# Autodesk Inventor assembly: Portalfraese_V2_Z-Axis
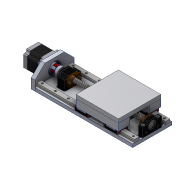
[picture p0: Inventor's stored thumbnail of the model, 180x180]
Saved by Autodesk Inventor 2016 (Build 200138000, 138)
## iProperties
Created: 2015-07-20
Part Number: Portalfraese_V2_Z-Axis
Document SubType Name: Assembly
Mass: 4544.64 g
Surface Area: 3288.98 cm^2
Volume: 1436.27 cm^3
Density: 3.16419 g/cm^3
## Documents named in this file (9)
- C:\Dropbox\Inventor\Projects\Portalfraese_V2_Z-Axis\Portalfraese_V2_Z-Axis.iam
- C:\Dropbox\Inventor\Projects\Portalfraese_V2_Z-Axis\Linearfuehrung Bosch Rexroth R0442.iam
- C:\Dropbox\Inventor\Projects\Portalfraese_V2_Z-Axis\ISSOKU_Ballscrew_D12x160_05_590104-13.iam
- C:\Dropbox\Inventor\Projects\Portalfraese_V2_Z-Axis\Grundplatte.ipt
- C:\Dropbox\Inventor\Projects\Portalfraese_V2_Z-Axis\Befestigungsplatte.ipt
- C:\Dropbox\Inventor\Projects\001_EK-Teile\Motor Nema 23.ipt
- C:\Dropbox\Inventor\Projects\Portalfraese_V2_Z-Axis\Motorhalterung.ipt
- C:\Dropbox\Inventor\Projects\Portalfraese_V2_Z-Axis\Distanzblock.ipt
- C:\Dropbox\Inventor\Projects\Portalfraese_V2_Z-Axis\Klauenkupplung.ipt
## Components (10 placed, 8 different names)
1. ISSOKU_Ballscrew_D12x160_05_590104-13:1 [sub-assembly] — Flush:1, Flush:2, Flush:6, Flush:7, Mate:3, Mate:5, Mate:6, Mate:7, Mate:8, Insert:1
2. Linearfuehrung Bosch Rexroth R0442:1 [sub-assembly] — Flush:1, Flush:3, Mate:1, Mate:2, Flush:4, Flush:5, Flush:6, Flush:7, Mate:4, Flush:8, Flush:9, Mate:12
3. Linearfuehrung Bosch Rexroth R0442:2 [sub-assembly] — Flush:2, Flush:3, Mate:2, Flush:4, Flush:5, Mate:13
4. Grundplatte:1 — Mate:3, Mate:4, Flush:8, Mate:5, Angle:1, Mate:10, Flush:10
5. Befestigungsplatte:1 — Mate:6, Flush:9, Mate:7, Flush:11, Flush:12, Flush:13, Flush:14
6. Motor Nema 23:1 — Mate:8, Angle:1, Mate:11, Mate:14
7. Motorhalterung:1 — Mate:10, Mate:11, Flush:10, Mate:14
8. Distanzblock:1 — Mate:12, Flush:11, Flush:12
9. Distanzblock:2 — Flush:13, Flush:14, Mate:13
10. Klauenkupplung:1 — Insert:1
## Relationships (29: Flush 14, Mate 13, Angle 1, Insert 1)
- Flush:1: ISSOKU_Ballscrew_D12x160_05_590104-13:1 ↔ Linearfuehrung Bosch Rexroth R0442:1
- Flush:2: ISSOKU_Ballscrew_D12x160_05_590104-13:1 ↔ Linearfuehrung Bosch Rexroth R0442:2
- Flush:3: Linearfuehrung Bosch Rexroth R0442:1 ↔ Linearfuehrung Bosch Rexroth R0442:2
- Mate:1 (40 mm): Linearfuehrung Bosch Rexroth R0442:1
- Mate:2 (80 mm): Linearfuehrung Bosch Rexroth R0442:1 ↔ Linearfuehrung Bosch Rexroth R0442:2
- Flush:4: Linearfuehrung Bosch Rexroth R0442:1 ↔ Linearfuehrung Bosch Rexroth R0442:2
- Flush:5: Linearfuehrung Bosch Rexroth R0442:1 ↔ Linearfuehrung Bosch Rexroth R0442:2
- Flush:6 (30 mm): ISSOKU_Ballscrew_D12x160_05_590104-13:1 ↔ Linearfuehrung Bosch Rexroth R0442:1
- Flush:7 (-60 mm): ISSOKU_Ballscrew_D12x160_05_590104-13:1 ↔ Linearfuehrung Bosch Rexroth R0442:1
- Mate:3: ISSOKU_Ballscrew_D12x160_05_590104-13:1 ↔ Grundplatte:1
- Mate:4: Linearfuehrung Bosch Rexroth R0442:1 ↔ Grundplatte:1
- Flush:8: Linearfuehrung Bosch Rexroth R0442:1 ↔ Grundplatte:1
- Mate:5 (3 mm): ISSOKU_Ballscrew_D12x160_05_590104-13:1 ↔ Grundplatte:1
- Mate:6 (-2 mm): ISSOKU_Ballscrew_D12x160_05_590104-13:1 ↔ Befestigungsplatte:1
- Flush:9 (-4 mm): Linearfuehrung Bosch Rexroth R0442:1 ↔ Befestigungsplatte:1
- Mate:7: ISSOKU_Ballscrew_D12x160_05_590104-13:1 ↔ Befestigungsplatte:1
- Mate:8: ISSOKU_Ballscrew_D12x160_05_590104-13:1 ↔ Motor Nema 23:1
- Angle:1 (0 deg): Grundplatte:1 ↔ Motor Nema 23:1
- Mate:10: Grundplatte:1 ↔ Motorhalterung:1
- Mate:11: Motor Nema 23:1 ↔ Motorhalterung:1
- Flush:10: Grundplatte:1 ↔ Motorhalterung:1
- Mate:12: Linearfuehrung Bosch Rexroth R0442:1 ↔ Distanzblock:1
- Flush:11: Befestigungsplatte:1 ↔ Distanzblock:1
- Flush:12: Befestigungsplatte:1 ↔ Distanzblock:1
- Flush:13: Befestigungsplatte:1 ↔ Distanzblock:2
- Flush:14: Befestigungsplatte:1 ↔ Distanzblock:2
- Mate:13: Linearfuehrung Bosch Rexroth R0442:2 ↔ Distanzblock:2
- Insert:1 (1.5 mm): ISSOKU_Ballscrew_D12x160_05_590104-13:1 ↔ Klauenkupplung:1
- Mate:14: Motor Nema 23:1 ↔ Motorhalterung:1
